# Autodesk Inventor assembly: yagi_Front
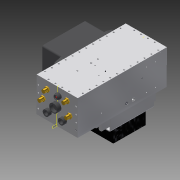
[picture p0: Inventor's stored thumbnail of the model, 180x180]
Saved by Autodesk Inventor 2014 (Build 180170000, 170)
## iProperties
Created: 2015-01-07
Part Number: yagi_Front
Document SubType Name: Assembly
Designer: Owner
Author: Owner
## Documents named in this file (66)
- C:\Users\Owner\Documents\APC\FrontEnd\IAM\Yagi\yagi_Front.iam
- C:\Users\Owner\Documents\APC\FrontEnd\IAM\Yagi\YagiBoard.iam
- C:\Users\Owner\Documents\APC\FrontEnd\IAM\Common\Yagi_BaseFrame.ipt
- C:\Users\Owner\Documents\APC\FrontEnd\IAM\Yagi\Yagi_Front_BackPlate.ipt
- C:\Users\Owner\Documents\APC\FrontEnd\IAM\Common\LED_Inset.ipt
- C:\Users\Owner\Documents\APC\FrontEnd\IAM\Common\BiglConnector.ipt
- C:\Users\Owner\Documents\APC\FrontEnd\IAM\Common\SmallConnector.ipt
- C:\Users\Owner\Documents\APC\FrontEnd\IAM\Yagi\SMA_Bulkhead.ipt
- C:\Users\Owner\Documents\APC\FrontEnd\IAM\Common\InjectorBoard2.iam
- C:\Users\Owner\Documents\APC\FrontEnd\IAM\Common\Peltier.ipt
- C:\Users\Owner\Documents\APC\FrontEnd\IAM\Common\PeltierPower.iam
- C:\Users\Owner\Documents\APC\FrontEnd\IAM\Common\Fan60.ipt
- C:\Users\Owner\Documents\APC\FrontEnd\IAM\Common\HeatSink60.ipt
- C:\Users\Owner\Documents\APC\FrontEnd\IAM\Common\NEAMBox.ipt
- C:\Users\Owner\Documents\APC\FrontEnd\IAM\Yagi\ColdFingerBase.ipt
- C:\Users\Owner\Documents\APC\FrontEnd\IAM\Yagi\ColdFingerStem.ipt
- C:\Users\Owner\Documents\APC\FrontEnd\IAM\Yagi\PeltierThermalSpacer.ipt
- C:\Users\Owner\Documents\APC\FrontEnd\IAM\Yagi\PeltierHeatSinkMount.ipt
- C:\Users\Owner\Documents\APC\FrontEnd\IAM\Yagi\YagiTop.ipt
- C:\Users\Owner\Documents\APC\FrontEnd\IAM\Common\PeltierController.iam
- C:\Users\Owner\Documents\APC\FrontEnd\IAM\Yagi\CavitySplitter.ipt
- C:\Users\Owner\Documents\APC\FrontEnd\IAM\Common\AmpPS.iam
- C:\Users\Owner\Documents\APC\FrontEnd\IAM\Yagi\YagiFanMetal.ipt
- C:\Users\Owner\Documents\APC\FrontEnd\IAM\Yagi\yagi_Front\Design Accelerator\Bolted Connection1.iam
- C:\Users\Owner\Documents\APC\FrontEnd\IAM\Yagi\yagi_Front\Design Accelerator\Bolted Connection2.iam
- C:\Users\Owner\Documents\APC\FrontEnd\IAM\Yagi\yagi_Front\Design Accelerator\Bolted Connection3.iam
- C:\Users\Owner\Documents\APC\FrontEnd\IAM\Yagi\yagi_Front\Design Accelerator\Bolted Connection4.iam
- C:\Users\Owner\Documents\APC\FrontEnd\IAM\Yagi\yagi_Front\Design Accelerator\Bolted Connection5.iam
- C:\Users\Owner\Documents\APC\FrontEnd\IAM\Yagi\yagi_Front\Design Accelerator\Bolted Connection6.iam
- C:\Users\Owner\Documents\APC\FrontEnd\IAM\Yagi\yagi_Front\Design Accelerator\Bolted Connection7.iam
- C:\Users\Owner\Documents\APC\FrontEnd\IAM\Yagi\yagi_Front\Design Accelerator\Bolted Connection8.iam
- C:\Users\Owner\Documents\APC\FrontEnd\IAM\Yagi\yagi_Front\Design Accelerator\Bolted Connection9.iam
- C:\Users\Owner\Documents\APC\FrontEnd\IAM\Dish\YagiFrontPanel.ipt
- C:\Users\Owner\Documents\APC\FrontEnd\IAM\Yagi\yagi_Front\Design Accelerator\Bolted Connection10.iam
- C:\Users\Owner\Documents\APC\FrontEnd\IAM\Dish\YagiBottom.ipt
- C:\Users\Owner\Documents\APC\FrontEnd\IAM\Yagi\yagi_Front\Design Accelerator\Bolted Connection11.iam
- C:\Users\Owner\Documents\APC\FrontEnd\IAM\Yagi\yagi_Front\Design Accelerator\Bolted Connection12.iam
- C:\Users\Owner\Documents\APC\FrontEnd\IAM\Yagi\yagi_Front\Design Accelerator\Bolted Connection13.iam
- C:\Users\Owner\Documents\APC\FrontEnd\IAM\Yagi\yagi_Front\Design Accelerator\Bolted Connection14.iam
- C:\Users\Owner\Documents\APC\FrontEnd\IAM\Yagi\yagi_Front\Design Accelerator\Bolted Connection15.iam
- C:\Users\Owner\Documents\APC\FrontEnd\IAM\Yagi\yagi_Front\Design Accelerator\Bolted Connection16.iam
- C:\Users\Owner\Documents\APC\FrontEnd\IAM\Yagi\yagi_Front\Design Accelerator\Bolted Connection17.iam
- C:\Users\Owner\Documents\APC\FrontEnd\IAM\Yagi\yagi_Front\Design Accelerator\Bolted Connection18.iam
- C:\Users\Owner\Documents\APC\FrontEnd\IAM\Yagi\yagi_Front\Design Accelerator\Bolted Connection19.iam
- C:\Users\Owner\Documents\APC\FrontEnd\IAM\Yagi\yagi_Front\Design Accelerator\Bolted Connection20.iam
- C:\Users\Owner\Documents\APC\FrontEnd\IAM\Yagi\yagi_Front\Design Accelerator\Bolted Connection21.iam
- C:\Users\Owner\Documents\APC\FrontEnd\IAM\Yagi\yagi_Front\Design Accelerator\Bolted Connection22.iam
- C:\Users\Owner\Documents\APC\FrontEnd\IAM\Yagi\yagi_Front\Design Accelerator\Bolted Connection23.iam
- C:\Users\Owner\Documents\APC\FrontEnd\IAM\Yagi\yagi_Front\Design Accelerator\Bolted Connection24.iam
- C:\Users\Owner\Documents\APC\FrontEnd\IAM\Yagi\yagi_Front\Design Accelerator\Bolted Connection25.iam
- C:\Users\Owner\Documents\APC\FrontEnd\IAM\Yagi\yagi_Front\Design Accelerator\Bolted Connection26.iam
- C:\Users\Owner\Documents\APC\FrontEnd\IAM\Yagi\YagiPSUSide.ipt
- C:\Users\Owner\Documents\APC\FrontEnd\IAM\Yagi\yagi_Front\Design Accelerator\Bolted Connection27.iam
- C:\Users\Owner\Documents\APC\FrontEnd\IAM\Yagi\yagi_Front\Design Accelerator\Bolted Connection28.iam
- C:\Users\Owner\Documents\APC\FrontEnd\IAM\Yagi\yagi_Front\Design Accelerator\Bolted Connection29.iam
- C:\Users\Owner\Documents\APC\FrontEnd\IAM\Yagi\yagi_Front\Design Accelerator\Bolted Connection30.iam
- C:\Users\Owner\Documents\APC\FrontEnd\IAM\Yagi\yagi_Front\Design Accelerator\Bolted Connection31.iam
- C:\Users\Owner\Documents\APC\FrontEnd\IAM\Yagi\yagi_Front\Design Accelerator\Bolted Connection32.iam
- C:\Users\Owner\Documents\APC\FrontEnd\IAM\Yagi\yagi_Front\Design Accelerator\Bolted Connection33.iam
- C:\Users\Owner\Documents\APC\FrontEnd\IAM\Yagi\yagi_Front\Design Accelerator\Bolted Connection34.iam
- C:\Users\Owner\Documents\APC\FrontEnd\IAM\Yagi\yagi_Front\Design Accelerator\Bolted Connection35.iam
- C:\Users\Owner\Documents\APC\FrontEnd\IAM\Yagi\yagi_Front\Design Accelerator\Bolted Connection36.iam
- C:\Users\Owner\Documents\APC\FrontEnd\IAM\Yagi\yagi_Front\Design Accelerator\Bolted Connection37.iam
- C:\Users\Owner\Documents\APC\FrontEnd\IAM\Yagi\yagi_Front\Design Accelerator\Bolted Connection38.iam
- C:\Users\Owner\Documents\APC\FrontEnd\IAM\Yagi\yagi_Front\Design Accelerator\Bolted Connection39.iam
- C:\Users\Owner\Documents\APC\FrontEnd\IAM\Yagi\yagi_Front\Design Accelerator\Bolted Connection40.iam
## Components (70 placed, 26 different names)
1. YagiBoard:1 [sub-assembly] — Mate:176, Flush:48, Mate:112, Mate:113, Mate:201, Mate:202, Mate:203, Mate:204, Mate:205, Mate:206, Mate:207, Mate:208, Mate:209, Mate:210, Mate:211, Mate:212
2. Yagi_BaseFrame:2 — Flush:22, Flush:57, Flush:58, Flush:61, Mate:174, Mate:175, Mate:177, Mate:178
3. Yagi_Front_BackPlate:1 — Mate:22, Mate:25, Mate:26, Mate:27, Mate:28, Mate:29, Mate:30, Mate:31, Mate:39, Mate:40, Mate:41, Mate:42, Mate:43, Mate:44, Mate:45, Mate:46, Angle:2, Angle:3, Angle:4, Angle:5, Flush:22, Flush:41, Flush:42, Flush:59, Flush:60, Mate:150, Flush:64, Flush:66, Mate:175, Mate:187, Mate:188, Mate:215, Mate:216
4. LED_Inset:2 — Mate:22, Mate:25
5. BiglConnector:1 — Mate:26, Mate:31
6. SmallConnector:1 — Mate:27, Mate:30
7. SmallConnector:2 — Mate:28, Mate:29
8. SMA_Bulkhead:1 — Mate:40, Mate:45, Angle:3
9. SMA_Bulkhead:2 — Mate:39, Mate:46, Angle:2
10. SMA_Bulkhead:3 — Mate:41, Mate:44, Angle:4
11. SMA_Bulkhead:4 — Mate:42, Mate:43, Angle:5
12. YagiBoard:2 [sub-assembly] — Mate:114, Mate:115, Mate:173, Mate:217, Mate:218, Mate:219, Mate:220, Mate:221, Mate:222, Mate:223, Mate:224, Mate:225, Mate:226, Mate:227, Mate:228
13. InjectorBoard2:1 [sub-assembly] — Mate:63, Flush:48, Mate:65, Flush:50, Mate:195, Mate:196, Mate:197, Mate:198, Mate:199, Mate:200
14. Peltier:1 — Flush:28, Flush:29, Flush:30, Flush:33, Flush:34, Flush:35
15. ColdFingerBase:1 — Flush:28, Flush:29, Flush:30, Mate:55, Flush:31, Mate:58, Mate:159
16. ColdFingerStem:1 — Mate:55, Flush:31, Mate:58
17. PeltierThermalSpacer:1 — Flush:33, Flush:34, Flush:35, Mate:56, Mate:67, Mate:68, Mate:71
18. YagiTop:1 — Flush:41, Flush:42, Mate:57, Flush:44, Flush:45, Mate:61, Flush:47, Mate:67, Mate:69, Flush:53, Flush:62, Mate:151, Flush:63, Mate:156, Mate:157, Flush:64, Mate:179, Mate:180, Mate:181, Mate:182, Mate:185, Mate:186, Mate:245, Mate:246
19. CavitySplitter:1 — Mate:61, Mate:63, Flush:47, Mate:64, Flush:49, Flush:50, Flush:67
20. AmpPS:1 [sub-assembly] — Mate:64, Flush:49, Mate:65, Mate:116, Mate:117, Mate:118, Mate:119
21. Bolted Connection:5 [sub-assembly] — Mate:177, Mate:178
22. Bolted Connection:6 [sub-assembly] — Mate:179, Mate:180
23. Bolted Connection:7 [sub-assembly] — Mate:181, Mate:182
24. Bolted Connection:8 [sub-assembly] — Mate:245, Mate:246
25. Bolted Connection:9 [sub-assembly] — Mate:187, Mate:188
26. YagiFrontPanel:1 — Flush:57, Flush:58, Mate:112, Mate:113, Mate:114, Mate:115, Flush:62, Mate:173, Mate:176, Mate:191, Mate:192, Mate:213, Mate:214
27. Bolted Connection:10 [sub-assembly] — Mate:185, Mate:186
28. YagiBottom:1 — Flush:59, Flush:60, Flush:61, Mate:126, Mate:127, Mate:136, Mate:137, Flush:65, Mate:174, Flush:67, Mate:189, Mate:190, Mate:193, Mate:194
29. YagiPSUSide:1 — Mate:150, Mate:151, Flush:63, Mate:158, Mate:172
30. Bolted Connection:11 [sub-assembly] — Mate:126, Mate:127
31. Bolted Connection:12 [sub-assembly] — Mate:189, Mate:190
32. Bolted Connection:13 [sub-assembly] — Mate:191, Mate:192
33. Bolted Connection:14 [sub-assembly] — Mate:136, Mate:137
34. Bolted Connection:15 [sub-assembly] — Mate:193, Mate:194
35. Bolted Connection:16 [sub-assembly] — Mate:116, Mate:117
36. Bolted Connection:17 [sub-assembly] — Mate:118, Mate:119
37. Bolted Connection:18 [sub-assembly] — Mate:195, Mate:196
38. Bolted Connection:19 [sub-assembly] — Mate:197, Mate:198
39. Bolted Connection:20 [sub-assembly] — Mate:199, Mate:200
40. Bolted Connection:21 [sub-assembly] — Mate:201, Mate:202
41. Bolted Connection:22 [sub-assembly] — Mate:203, Mate:204
42. Bolted Connection:23 [sub-assembly] — Mate:205, Mate:206
43. Bolted Connection:24 [sub-assembly] — Mate:207, Mate:208
44. Bolted Connection:25 [sub-assembly] — Mate:209, Mate:210
45. Bolted Connection:26 [sub-assembly] — Mate:211, Mate:212
46. Bolted Connection:27 [sub-assembly] — Mate:213, Mate:214
47. Bolted Connection:28 [sub-assembly] — Mate:215, Mate:216
48. Bolted Connection:29 [sub-assembly] — Mate:156, Mate:157
49. Bolted Connection:30 [sub-assembly] — Mate:158, Mate:159
50. Bolted Connection:31 [sub-assembly] — Mate:217, Mate:218
51. Bolted Connection:32 [sub-assembly] — Mate:219, Mate:220
52. Bolted Connection:33 [sub-assembly] — Mate:221, Mate:222
53. Bolted Connection:34 [sub-assembly] — Mate:223, Mate:224
54. Bolted Connection:35 [sub-assembly] — Mate:225, Mate:226
55. Bolted Connection:36 [sub-assembly] — Mate:227, Mate:228
56. Bolted Connection:37 [sub-assembly] — Mate:237, Mate:238
57. Bolted Connection:38 [sub-assembly] — Mate:239, Mate:240
58. Bolted Connection:39 [sub-assembly] — Mate:241, Mate:242
59. Bolted Connection:40 [sub-assembly] — Mate:243, Mate:244
60. PeltierPower:1 [sub-assembly] — Mate:51, Mate:52, Mate:53
61. NEAMBox:1 — Mate:51, Mate:52, Mate:53, Mate:59, Mate:60, Mate:172, Flush:65, Flush:66, Mate:237, Mate:238, Mate:239, Mate:240, Mate:241, Mate:242, Mate:243, Mate:244
62. PeltierController:1 [sub-assembly] — Mate:59, Mate:60
63. HeatSink60:1 — Mate:56, Flush:38, Flush:54, Flush:55
64. PeltierHeatSinkMount:1 — Flush:38, Mate:57, Flush:44, Flush:45, Mate:68
65. Bolted Connection:1 [sub-assembly] — Mate:229, Mate:230
66. Bolted Connection:2 [sub-assembly] — Mate:231, Mate:232
67. Bolted Connection:3 [sub-assembly] — Mate:233, Mate:234
68. Bolted Connection:4 [sub-assembly] — Mate:235, Mate:236
69. YagiFanMetal:1 — Mate:66, Flush:52, Mate:69, Flush:53, Mate:70, Mate:71, Flush:54
70. Fan60:1 — Mate:66, Flush:52, Mate:70, Flush:55, Mate:229, Mate:230, Mate:231, Mate:232, Mate:233, Mate:234, Mate:235, Mate:236
## Relationships (162: Mate 126, Flush 32, Angle 4)
- Mate:22: Yagi_Front_BackPlate:1 ↔ LED_Inset:2
- Mate:25: Yagi_Front_BackPlate:1 ↔ LED_Inset:2
- Mate:26: Yagi_Front_BackPlate:1 ↔ BiglConnector:1
- Mate:27: Yagi_Front_BackPlate:1 ↔ SmallConnector:1
- Mate:28: Yagi_Front_BackPlate:1 ↔ SmallConnector:2
- Mate:29: Yagi_Front_BackPlate:1 ↔ SmallConnector:2
- Mate:30: Yagi_Front_BackPlate:1 ↔ SmallConnector:1
- Mate:31: Yagi_Front_BackPlate:1 ↔ BiglConnector:1
- Mate:39: Yagi_Front_BackPlate:1 ↔ SMA_Bulkhead:2
- Mate:40: Yagi_Front_BackPlate:1 ↔ SMA_Bulkhead:1
- Mate:41: Yagi_Front_BackPlate:1 ↔ SMA_Bulkhead:3
- Mate:42: Yagi_Front_BackPlate:1 ↔ SMA_Bulkhead:4
- Mate:43: Yagi_Front_BackPlate:1 ↔ SMA_Bulkhead:4
- Mate:44: Yagi_Front_BackPlate:1 ↔ SMA_Bulkhead:3
- Mate:45: Yagi_Front_BackPlate:1 ↔ SMA_Bulkhead:1
- Mate:46: Yagi_Front_BackPlate:1 ↔ SMA_Bulkhead:2
- Angle:2 (0 deg): Yagi_Front_BackPlate:1 ↔ SMA_Bulkhead:2
- Angle:3 (0 deg): Yagi_Front_BackPlate:1 ↔ SMA_Bulkhead:1
- Angle:4 (0 deg): Yagi_Front_BackPlate:1 ↔ SMA_Bulkhead:3
- Angle:5 (0 deg): Yagi_Front_BackPlate:1 ↔ SMA_Bulkhead:4
- Mate:176: YagiBoard:1 ↔ YagiFrontPanel:1
- Flush:22: Yagi_BaseFrame:2 ↔ Yagi_Front_BackPlate:1
- Mate:51: PeltierPower:1 ↔ NEAMBox:1
- Mate:52 (6.35 mm): PeltierPower:1 ↔ NEAMBox:1
- Mate:53 (3.175 mm): PeltierPower:1 ↔ NEAMBox:1
- Flush:28: Peltier:1 ↔ ColdFingerBase:1
- Flush:29: Peltier:1 ↔ ColdFingerBase:1
- Flush:30: Peltier:1 ↔ ColdFingerBase:1
- Mate:55: ColdFingerBase:1 ↔ ColdFingerStem:1
- Flush:31: ColdFingerBase:1 ↔ ColdFingerStem:1
- Mate:58: ColdFingerBase:1 ↔ ColdFingerStem:1
- Flush:33: Peltier:1 ↔ PeltierThermalSpacer:1
- Flush:34: Peltier:1 ↔ PeltierThermalSpacer:1
- Flush:35: Peltier:1 ↔ PeltierThermalSpacer:1
- Mate:56: PeltierThermalSpacer:1 ↔ HeatSink60:1
- Flush:38: HeatSink60:1 ↔ PeltierHeatSinkMount:1
- Flush:41: Yagi_Front_BackPlate:1 ↔ YagiTop:1
- Flush:42: Yagi_Front_BackPlate:1 ↔ YagiTop:1
- Mate:57: YagiTop:1 ↔ PeltierHeatSinkMount:1
- Flush:44: YagiTop:1 ↔ PeltierHeatSinkMount:1
- Flush:45: YagiTop:1 ↔ PeltierHeatSinkMount:1
- Mate:59: NEAMBox:1 ↔ PeltierController:1
- Mate:60 (6.35 mm): NEAMBox:1 ↔ PeltierController:1
- Mate:61: YagiTop:1 ↔ CavitySplitter:1
- Mate:63: InjectorBoard2:1 ↔ CavitySplitter:1
- Flush:47: YagiTop:1 ↔ CavitySplitter:1
- Flush:48: YagiBoard:1 ↔ InjectorBoard2:1
- Mate:64 (1.5875 mm): CavitySplitter:1 ↔ AmpPS:1
- Flush:49: CavitySplitter:1 ↔ AmpPS:1
- Mate:65 (1.5875 mm): InjectorBoard2:1 ↔ AmpPS:1
- Flush:50 (3.175 mm): InjectorBoard2:1 ↔ CavitySplitter:1
- Mate:66: YagiFanMetal:1 ↔ Fan60:1
- Flush:52 (10 mm): YagiFanMetal:1 ↔ Fan60:1
- Mate:67 (2.5 mm): PeltierThermalSpacer:1 ↔ YagiTop:1
- Mate:68 (2.5 mm): PeltierThermalSpacer:1 ↔ PeltierHeatSinkMount:1
- Mate:69: YagiTop:1 ↔ YagiFanMetal:1
- Flush:53 (3.175 mm): YagiTop:1 ↔ YagiFanMetal:1
- Mate:70 (-10 mm): YagiFanMetal:1 ↔ Fan60:1
- Mate:71: PeltierThermalSpacer:1 ↔ YagiFanMetal:1
- Flush:54 (-10 mm): HeatSink60:1 ↔ YagiFanMetal:1
- Flush:55 (-2 mm): HeatSink60:1 ↔ Fan60:1
- Flush:57: Yagi_BaseFrame:2 ↔ YagiFrontPanel:1
- Flush:58: Yagi_BaseFrame:2 ↔ YagiFrontPanel:1
- Flush:59: Yagi_Front_BackPlate:1 ↔ YagiBottom:1
- Flush:60: Yagi_Front_BackPlate:1 ↔ YagiBottom:1
- Flush:61: Yagi_BaseFrame:2 ↔ YagiBottom:1
- Mate:112: YagiBoard:1 ↔ YagiFrontPanel:1
- Mate:113: YagiBoard:1 ↔ YagiFrontPanel:1
- Mate:114: YagiBoard:2 ↔ YagiFrontPanel:1
- Mate:115: YagiBoard:2 ↔ YagiFrontPanel:1
- Mate:116: AmpPS:1 ↔ Bolted Connection:16
- Mate:117: AmpPS:1 ↔ Bolted Connection:16
- Mate:118: AmpPS:1 ↔ Bolted Connection:17
- Mate:119: AmpPS:1 ↔ Bolted Connection:17
- Flush:62: YagiTop:1 ↔ YagiFrontPanel:1
- Mate:126: YagiBottom:1 ↔ Bolted Connection:11
- Mate:127: YagiBottom:1 ↔ Bolted Connection:11
- Mate:136: YagiBottom:1 ↔ Bolted Connection:14
- Mate:137: YagiBottom:1 ↔ Bolted Connection:14
- Mate:150: Yagi_Front_BackPlate:1 ↔ YagiPSUSide:1
- Mate:151: YagiTop:1 ↔ YagiPSUSide:1
- Flush:63: YagiTop:1 ↔ YagiPSUSide:1
- Mate:156: YagiTop:1 ↔ Bolted Connection:29
- Mate:157: YagiTop:1 ↔ Bolted Connection:29
- Mate:158: YagiPSUSide:1 ↔ Bolted Connection:30
- Mate:159: ColdFingerBase:1 ↔ Bolted Connection:30
- Mate:172: YagiPSUSide:1 ↔ NEAMBox:1
- Flush:64: Yagi_Front_BackPlate:1 ↔ YagiTop:1
- Flush:65: YagiBottom:1 ↔ NEAMBox:1
- Flush:66 (38.1 mm): Yagi_Front_BackPlate:1 ↔ NEAMBox:1
- Mate:173: YagiBoard:2 ↔ YagiFrontPanel:1
- Mate:174: Yagi_BaseFrame:2 ↔ YagiBottom:1
- Mate:175: Yagi_BaseFrame:2 ↔ Yagi_Front_BackPlate:1
- Flush:67 (28.575 mm): CavitySplitter:1 ↔ YagiBottom:1
- Mate:177: Yagi_BaseFrame:2 ↔ Bolted Connection:5
- Mate:178: Yagi_BaseFrame:2 ↔ Bolted Connection:5
- Mate:179: YagiTop:1 ↔ Bolted Connection:6
- Mate:180: YagiTop:1 ↔ Bolted Connection:6
- Mate:181: YagiTop:1 ↔ Bolted Connection:7
- Mate:182: YagiTop:1 ↔ Bolted Connection:7
- Mate:185: YagiTop:1 ↔ Bolted Connection:10
- Mate:186: YagiTop:1 ↔ Bolted Connection:10
- Mate:187: Yagi_Front_BackPlate:1 ↔ Bolted Connection:9
- Mate:188: Yagi_Front_BackPlate:1 ↔ Bolted Connection:9
- Mate:189: YagiBottom:1 ↔ Bolted Connection:12
- Mate:190: YagiBottom:1 ↔ Bolted Connection:12
- Mate:191: YagiFrontPanel:1 ↔ Bolted Connection:13
- Mate:192: YagiFrontPanel:1 ↔ Bolted Connection:13
- Mate:193: YagiBottom:1 ↔ Bolted Connection:15
- Mate:194: YagiBottom:1 ↔ Bolted Connection:15
- Mate:195: InjectorBoard2:1 ↔ Bolted Connection:18
- Mate:196: InjectorBoard2:1 ↔ Bolted Connection:18
- Mate:197: InjectorBoard2:1 ↔ Bolted Connection:19
- Mate:198: InjectorBoard2:1 ↔ Bolted Connection:19
- Mate:199: InjectorBoard2:1 ↔ Bolted Connection:20
- Mate:200: InjectorBoard2:1 ↔ Bolted Connection:20
- Mate:201: YagiBoard:1 ↔ Bolted Connection:21
- Mate:202: YagiBoard:1 ↔ Bolted Connection:21
- Mate:203: YagiBoard:1 ↔ Bolted Connection:22
- Mate:204: YagiBoard:1 ↔ Bolted Connection:22
- Mate:205: YagiBoard:1 ↔ Bolted Connection:23
- Mate:206: YagiBoard:1 ↔ Bolted Connection:23
- Mate:207: YagiBoard:1 ↔ Bolted Connection:24
- Mate:208: YagiBoard:1 ↔ Bolted Connection:24
- Mate:209: YagiBoard:1 ↔ Bolted Connection:25
- Mate:210: YagiBoard:1 ↔ Bolted Connection:25
- Mate:211: YagiBoard:1 ↔ Bolted Connection:26
- Mate:212: YagiBoard:1 ↔ Bolted Connection:26
- Mate:213: YagiFrontPanel:1 ↔ Bolted Connection:27
- Mate:214: YagiFrontPanel:1 ↔ Bolted Connection:27
- Mate:215: Yagi_Front_BackPlate:1 ↔ Bolted Connection:28
- Mate:216: Yagi_Front_BackPlate:1 ↔ Bolted Connection:28
- Mate:217: YagiBoard:2 ↔ Bolted Connection:31
- Mate:218: YagiBoard:2 ↔ Bolted Connection:31
- Mate:219: YagiBoard:2 ↔ Bolted Connection:32
- Mate:220: YagiBoard:2 ↔ Bolted Connection:32
- Mate:221: YagiBoard:2 ↔ Bolted Connection:33
- Mate:222: YagiBoard:2 ↔ Bolted Connection:33
- Mate:223: YagiBoard:2 ↔ Bolted Connection:34
- Mate:224: YagiBoard:2 ↔ Bolted Connection:34
- Mate:225: YagiBoard:2 ↔ Bolted Connection:35
- Mate:226: YagiBoard:2 ↔ Bolted Connection:35
- Mate:227: YagiBoard:2 ↔ Bolted Connection:36
- Mate:228: YagiBoard:2 ↔ Bolted Connection:36
- Mate:229: Bolted Connection:1 ↔ Fan60:1
- Mate:230: Bolted Connection:1 ↔ Fan60:1
- Mate:231: Bolted Connection:2 ↔ Fan60:1
- Mate:232: Bolted Connection:2 ↔ Fan60:1
- Mate:233: Bolted Connection:3 ↔ Fan60:1
- Mate:234: Bolted Connection:3 ↔ Fan60:1
- Mate:235: Bolted Connection:4 ↔ Fan60:1
- Mate:236: Bolted Connection:4 ↔ Fan60:1
- Mate:237: Bolted Connection:37 ↔ NEAMBox:1
- Mate:238: Bolted Connection:37 ↔ NEAMBox:1
- Mate:239: Bolted Connection:38 ↔ NEAMBox:1
- Mate:240: Bolted Connection:38 ↔ NEAMBox:1
- Mate:241: Bolted Connection:39 ↔ NEAMBox:1
- Mate:242: Bolted Connection:39 ↔ NEAMBox:1
- Mate:243: Bolted Connection:40 ↔ NEAMBox:1
- Mate:244: Bolted Connection:40 ↔ NEAMBox:1
- Mate:245: YagiTop:1 ↔ Bolted Connection:8
- Mate:246: YagiTop:1 ↔ Bolted Connection:8
